# Autodesk Inventor assembly: final
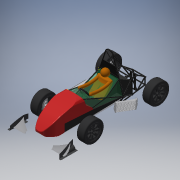
[picture p0: Inventor's stored thumbnail of the model, 180x180]
Saved by Autodesk Inventor 2018.1 (Build 221171000, 171)
## iProperties
Created: 2017-11-01
Part Number: final
Material: 一般
Document SubType Name: Assembly
Designer: kuwano
Author: kuwano
## Documents named in this file (3)
- D:\kuwano\Documents\Inventor\KITformula\KS-15_Aero_CAD\test\final.iam
- D:\kuwano\Documents\Inventor\KITformula\KS-15_Aero_CAD\ks-14_slow\KS-14_SLow_replace.iam
- D:\kuwano\Documents\Inventor\KITformula\KS-15_Aero_CAD\test\Assembly1.iam
## Components (2 placed, 2 different names)
1. KS-14_SLow_replace:1 [sub-assembly] — フラッシュ:1, フラッシュ:2, フラッシュ:3, フラッシュ:5, メイト:1
2. Assembly1:1 [sub-assembly] — フラッシュ:4, フラッシュ:5, メイト:1
## Relationships (6: Flush 5, Mate 1)
- フラッシュ:1 [Flush]: KS-14_SLow_replace:1
- フラッシュ:2 [Flush]: KS-14_SLow_replace:1
- フラッシュ:3 [Flush]: KS-14_SLow_replace:1
- フラッシュ:4 [Flush] (-250 mm): Assembly1:1
- フラッシュ:5 [Flush] (-10 mm): KS-14_SLow_replace:1 ↔ Assembly1:1
- メイト:1 [Mate] (400 mm): KS-14_SLow_replace:1 ↔ Assembly1:1
